# Autodesk Inventor assembly: distribucionDeCorte
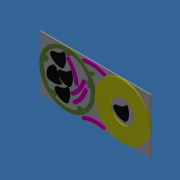
[picture p0: Inventor's stored thumbnail of the model, 180x180]
Saved by Autodesk Inventor 2014 (Build 180170000, 170)
## iProperties
Created: 2014-03-16
Part Number: distribucionDeCorte
Document SubType Name: Assembly
Designer: Lefo
Author: Lefo
## Documents named in this file (6)
- C:\Users\Lefo\Documents\Inventor\academy\something big\distribucionDeCorte.iam
- C:\Users\Lefo\Documents\Inventor\academy\petalo3.ipt
- C:\Users\Lefo\Documents\Inventor\academy\brazo.ipt
- C:\Users\Lefo\Documents\Inventor\academy\borde.ipt
- C:\Users\Lefo\Documents\Inventor\academy\something big\plancha.ipt
- C:\Users\Lefo\Documents\Inventor\academy\plancha1200x2400.ipt
## Components (13 placed, 5 different names)
1. petalo3:1 — Mate:9
2. petalo3:2 — Mate:10
3. petalo3:3 — Mate:12
4. petalo3:4 — Mate:11
5. petalo3:5 — Mate:8
6. brazo:1 — Mate:7
7. brazo:2 — Mate:6
8. brazo:3 — Mate:5
9. brazo:4 — Mate:4
10. brazo:5 — Mate:3
11. borde:1 — Mate:1
12. plancha:1 — Mate:2
13. plancha1200x2400:1 — Mate:1, Mate:2, Mate:3, Mate:4, Mate:5, Mate:6, Mate:7, Mate:8, Mate:9, Mate:10, Mate:11, Mate:12
## Relationships (12: Mate 12)
- Mate:1: borde:1 ↔ plancha1200x2400:1
- Mate:2: plancha:1 ↔ plancha1200x2400:1
- Mate:3: brazo:5 ↔ plancha1200x2400:1
- Mate:4: brazo:4 ↔ plancha1200x2400:1
- Mate:5: brazo:3 ↔ plancha1200x2400:1
- Mate:6: brazo:2 ↔ plancha1200x2400:1
- Mate:7: brazo:1 ↔ plancha1200x2400:1
- Mate:8: petalo3:5 ↔ plancha1200x2400:1
- Mate:9: petalo3:1 ↔ plancha1200x2400:1
- Mate:10: petalo3:2 ↔ plancha1200x2400:1
- Mate:11: petalo3:4 ↔ plancha1200x2400:1
- Mate:12: petalo3:3 ↔ plancha1200x2400:1
